# Autodesk Inventor assembly: reducer_unit
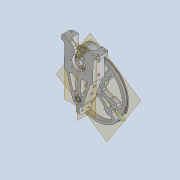
[picture p0: Inventor's stored thumbnail of the model, 180x180]
Saved by Autodesk Inventor 2020 (Build 240168000, 168)
## iProperties
Created: 2021-10-20
Part Number: reducer_unit
Document SubType Name: Assembly
Designer: Shuang Peng
Author: Shuang Peng
## Documents named in this file (6)
- D:\projects-3\torque fb tip\hardware\hapkit_1\reducer_unit.iam
- D:\projects-3\torque fb tip\hardware\hapkit_1\mot_27_ass.iam
- D:\projects-3\torque fb tip\hardware\hapkit_1\tendon_wh_1_mod.ipt
- D:\projects-3\torque fb tip\hardware\hapkit_1\driving_wheel_70.ipt
- D:\projects-3\torque fb tip\hardware\hapkit_1\mot_ss_1.ipt
- D:\projects-3\torque fb tip\hardware\hapkit_1\bearing_3_6_2.ipt
## Components (7 placed, 5 different names)
1. mot_27_ass:1 [sub-assembly] — Insert:1, Insert:2, Flush:2, Insert:4, Insert:5
2. tendon_wh_1_mod:1 — Insert:1, Insert:2, Flush:1, Tangent:1
3. driving_wheel_70:1 — Flush:1, Tangent:1, Insert:6, Insert:9
4. mot_ss_1:1 — Flush:2, Flush:3, Insert:4, Insert:5, Insert:6, Insert:7, Insert:8
5. bearing_3_6_2:1 — Insert:8
6. bearing_3_6_2:2 — Insert:7
7. bearing_3_6_2:3 — Insert:9
## Relationships (12: Insert 8, Flush 3, Tangent 1)
- Insert:1: mot_27_ass:1 ↔ tendon_wh_1_mod:1
- Insert:2: mot_27_ass:1 ↔ tendon_wh_1_mod:1
- Flush:1 (2 mm): tendon_wh_1_mod:1 ↔ driving_wheel_70:1
- Tangent:1 (0.7 mm): tendon_wh_1_mod:1 ↔ driving_wheel_70:1
- Flush:2: mot_27_ass:1 ↔ mot_ss_1:1
- Flush:3: mot_ss_1:1
- Insert:4: mot_27_ass:1 ↔ mot_ss_1:1
- Insert:5: mot_27_ass:1 ↔ mot_ss_1:1
- Insert:6: driving_wheel_70:1 ↔ mot_ss_1:1
- Insert:7: mot_ss_1:1 ↔ bearing_3_6_2:2
- Insert:8: mot_ss_1:1 ↔ bearing_3_6_2:1
- Insert:9: driving_wheel_70:1 ↔ bearing_3_6_2:3
